# Autodesk Inventor assembly: Assembly
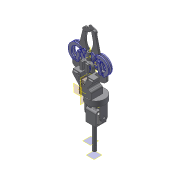
[picture p0: Inventor's stored thumbnail of the model, 180x180]
Saved by Autodesk Inventor 2018 (Build 220112000, 112)
## iProperties
Created: 2018-02-18
Part Number: Assembly
Document SubType Name: Assembly
Designer: Bardo91
Author: Bardo91
## Documents named in this file (11)
- E:\programming\hecatonquiros\cad_models\tools\gripper\serial_model_bearing_6DoF\Assembly_v2.iam
- E:\programming\hecatonquiros\cad_models\tools\gripper\serial_model_bearing_6DoF\attachment_arm2_grande_microsevometalico.ipt
- E:\programming\hecatonquiros\cad_models\tools\gripper\serial_model_bearing_6DoF\microservo_FT_2322.ipt
- E:\programming\hecatonquiros\cad_models\tools\gripper\serial_model_bearing_6DoF\middle_joint_microservo_metalico_v2.ipt
- E:\programming\hecatonquiros\cad_models\tools\gripper\serial_model_bearing_6DoF\base_gripper_v2.ipt
- E:\programming\hecatonquiros\cad_models\accesories\gripper\barra_triangulo.ipt
- E:\programming\hecatonquiros\cad_models\accesories\gripper\barragarra_pilar_3.ipt
- E:\programming\hecatonquiros\cad_models\tools\gripper\serial_model_0dof\gripper.ipt
- E:\programming\hecatonquiros\cad_models\tools\gripper\serial_model_6DoF\ScrewActuatorGripper.ipt
- E:\programming\hecatonquiros\cad_models\tools\gripper\serial_model_6DoF\ScrewActuatorGripperCenter.ipt
- E:\programming\hecatonquiros\cad_models\accesories\gripper\garra_pilar.ipt
## Components (19 placed, 10 different names)
1. attachment_arm2_grande_microsevometalico:1 — Mate:1, Mate:3, Mate:4, Mate:5, Mate:6
2. microservo_FT_2322:1 — Mate:1, Mate:3, Mate:4
3. middle_joint_microservo_metalico_v2:1 — Mate:5, Mate:6, Mate:7, Mate:8
4. base_gripper_v2:1 — Mate:7, Mate:8, Mate:9, Mate:11, Mate:12, Mate:13, Mate:14, Mate:15, Mate:16, Mate:25, Mate:26, Mate:27, Mate:28, Mate:47, Mate:48, Mate:50, Mate:52, Mate:53, Mate:54, Mate:57, Mate:58
5. microservo_FT_2322:2 — Mate:9, Mate:11, Mate:12, Mate:43
6. barra_triangulo:1 — Mate:41, Mate:46, Mate:51, Mate:56
7. barra_triangulo:2 — Mate:35, Mate:36, Mate:45, Mate:49, Mate:55
8. barragarra_pilar_3:1 — Mate:13, Mate:14, Mate:42
9. barragarra_pilar_3:2 — Mate:15, Mate:16, Mate:39, Mate:40
10. barragarra_pilar_3:3 — Mate:25, Mate:28, Mate:37
11. barragarra_pilar_3:4 — Mate:26, Mate:27, Mate:38
12. gripper:1 — Mate:39, Mate:40, Mate:41, Mate:42
13. gripper:2 — Mate:35, Mate:36, Mate:37, Mate:38
14. ScrewActuatorGripper:1 — Mate:43, Mate:44
15. ScrewActuatorGripperCenter:1 — Mate:44, Mate:45, Mate:46
16. garra_pilar:1 — Mate:47, Mate:48, Mate:49
17. garra_pilar:2 — Mate:50, Mate:51, Mate:52
18. garra_pilar:3 — Mate:53, Mate:55, Mate:58
19. garra_pilar:4 — Mate:54, Mate:56, Mate:57
## Relationships (42: Mate 42)
- Mate:1: attachment_arm2_grande_microsevometalico:1 ↔ microservo_FT_2322:1
- Mate:3: attachment_arm2_grande_microsevometalico:1 ↔ microservo_FT_2322:1
- Mate:4: attachment_arm2_grande_microsevometalico:1 ↔ microservo_FT_2322:1
- Mate:5: attachment_arm2_grande_microsevometalico:1 ↔ middle_joint_microservo_metalico_v2:1
- Mate:6: attachment_arm2_grande_microsevometalico:1 ↔ middle_joint_microservo_metalico_v2:1
- Mate:7: middle_joint_microservo_metalico_v2:1 ↔ base_gripper_v2:1
- Mate:8: middle_joint_microservo_metalico_v2:1 ↔ base_gripper_v2:1
- Mate:9: base_gripper_v2:1 ↔ microservo_FT_2322:2
- Mate:11: base_gripper_v2:1 ↔ microservo_FT_2322:2
- Mate:12: base_gripper_v2:1 ↔ microservo_FT_2322:2
- Mate:13: base_gripper_v2:1 ↔ barragarra_pilar_3:1
- Mate:14: base_gripper_v2:1 ↔ barragarra_pilar_3:1
- Mate:15: base_gripper_v2:1 ↔ barragarra_pilar_3:2
- Mate:16: base_gripper_v2:1 ↔ barragarra_pilar_3:2
- Mate:25: base_gripper_v2:1 ↔ barragarra_pilar_3:3
- Mate:26: base_gripper_v2:1 ↔ barragarra_pilar_3:4
- Mate:27: base_gripper_v2:1 ↔ barragarra_pilar_3:4
- Mate:28: base_gripper_v2:1 ↔ barragarra_pilar_3:3
- Mate:35: barra_triangulo:2 ↔ gripper:2
- Mate:36: barra_triangulo:2 ↔ gripper:2
- Mate:37: barragarra_pilar_3:3 ↔ gripper:2
- Mate:38: barragarra_pilar_3:4 ↔ gripper:2
- Mate:39: barragarra_pilar_3:2 ↔ gripper:1
- Mate:40: barragarra_pilar_3:2 ↔ gripper:1
- Mate:41: barra_triangulo:1 ↔ gripper:1
- Mate:42: barragarra_pilar_3:1 ↔ gripper:1
- Mate:43: microservo_FT_2322:2 ↔ ScrewActuatorGripper:1
- Mate:44: ScrewActuatorGripper:1 ↔ ScrewActuatorGripperCenter:1
- Mate:45: barra_triangulo:2 ↔ ScrewActuatorGripperCenter:1
- Mate:46: barra_triangulo:1 ↔ ScrewActuatorGripperCenter:1
- Mate:47: base_gripper_v2:1 ↔ garra_pilar:1
- Mate:48: base_gripper_v2:1 ↔ garra_pilar:1
- Mate:49: barra_triangulo:2 ↔ garra_pilar:1
- Mate:50: base_gripper_v2:1 ↔ garra_pilar:2
- Mate:51: barra_triangulo:1 ↔ garra_pilar:2
- Mate:52: base_gripper_v2:1 ↔ garra_pilar:2
- Mate:53: base_gripper_v2:1 ↔ garra_pilar:3
- Mate:54: base_gripper_v2:1 ↔ garra_pilar:4
- Mate:55: barra_triangulo:2 ↔ garra_pilar:3
- Mate:56: barra_triangulo:1 ↔ garra_pilar:4
- Mate:57: base_gripper_v2:1 ↔ garra_pilar:4
- Mate:58: base_gripper_v2:1 ↔ garra_pilar:3
